# Autodesk Inventor assembly: MicroUSB
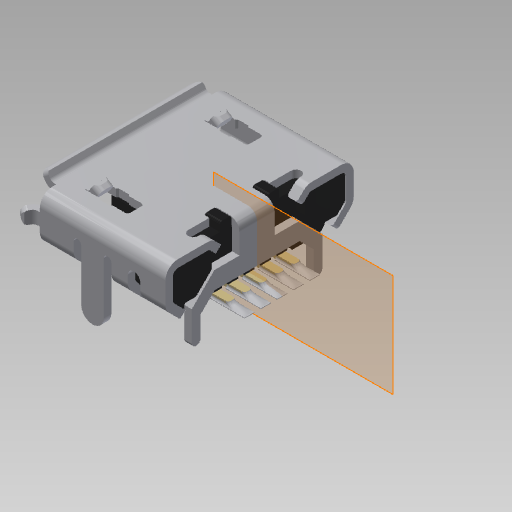
[picture p0: Inventor's stored thumbnail of the model, 512x512]
Saved by Autodesk Inventor 2020 (Build 240168000, 168)
## iProperties
Created: 2018-07-21
Part Number: MicroUSB
Description: STEP AP214
Document SubType Name: Assembly
Designer: amsmi
Preprocessor: SwSTEP 2.0
Title: TP4056 Charger Module.STEP
Author: M.B.I.
Revision Number: ANY
## Documents named in this file (2)
- C:\Users\Alex\Documents\Inventor Modeling\Legacy\Nanodevelopment Lab\Pirani Gauge\Final Readout\MicroUSB.iam
- C:\Users\Alex\Documents\Inventor Modeling\Legacy\Nanodevelopment Lab\Pirani Gauge\Final Readout\10_Micro USB-B SMD & pads.ipt
## Components (1 placed, 1 different names)
1. NAUO3
## Relationships (1: Flush 1)
- Flush:1 (0.338 mm)
